# Autodesk Inventor assembly: CheckBall
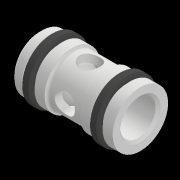
[picture p0: Inventor's stored thumbnail of the model, 180x180]
Saved by Autodesk Inventor 2021 (Build 250183000, 183)
## iProperties
Created: 2024-03-24
Part Number: CheckBall
Document SubType Name: Assembly
Designer: top10
Author: top10
## Documents named in this file (4)
- D:\Files\Graduation Project\V4_manfoulid\Workspaces\Workspace\CheckBall.iam
- D:\Files\Graduation Project\V4_manfoulid\Workspaces\Workspace\steelBall.ipt
- D:\Files\Graduation Project\V4_manfoulid\Workspaces\Workspace\checkBallValve.ipt
- D:\Files\Graduation Project\V4_manfoulid\Libraries\Content Center Files\en-US\DIN 3771(03)\DIN 3771 - 8.76 x 1.8 - N - NBR 70(4)11.88.ipt
## Components (4 placed, 3 different names)
1. steelBall:1
2. checkBallValve:1 — Mate:2, Mate:3
3. DIN 3771 hydraulic (External) 8.76 x 1.8 - N - NBR 70:1 — Mate:3
4. DIN 3771 hydraulic (External) 8.76 x 1.8 - N - NBR 70:2 — Mate:2
## Relationships (3: Mate 3)
- [Mate]: steelBall:1 ↔ checkBallValve:1
- Mate:2: checkBallValve:1 ↔ DIN 3771 hydraulic (External) 8.76 x 1.8 - N - NBR 70:2
- Mate:3: checkBallValve:1 ↔ DIN 3771 hydraulic (External) 8.76 x 1.8 - N - NBR 70:1
